# Autodesk Inventor assembly: main
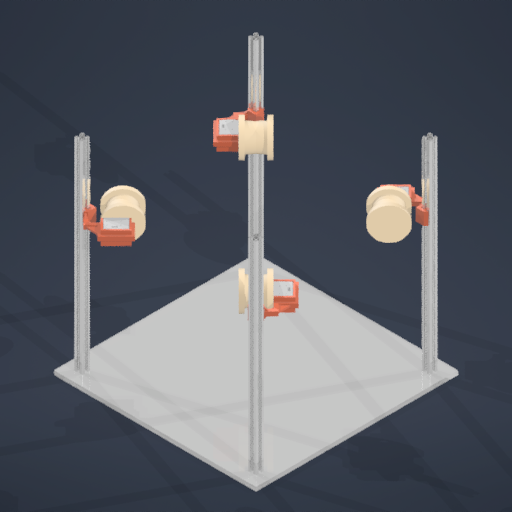
[picture p0: Inventor's stored thumbnail of the model, 512x512]
Saved by Autodesk Inventor 2026.2 (Build 302298010, 298A)
## iProperties
Created: 2026-02-11
Part Number: main
Document SubType Name: Assembly
Designer: Luke
Author: Luke
## Documents named in this file (3)
- C:\Users\Luke\OneDrive - Heriot-Watt University\Desktop\Robot Mech Sys\GroupProject\CAD\main.iam
- C:\Users\Luke\OneDrive - Heriot-Watt University\Desktop\Robot Mech Sys\GroupProject\CAD\parts\base.ipt
- C:\Users\Luke\OneDrive - Heriot-Watt University\Desktop\Robot Mech Sys\GroupProject\CAD\sub_assemblies\beam_sub_asssem.iam
## Components (5 placed, 2 different names)
1. base:1 — Mate:1, Mate:2, Mate:3, Flush:1, Flush:2
2. beam_sub_asssem:1 [sub-assembly] — Mate:1, Mate:2, Mate:3
3. beam_sub_asssem:2 [sub-assembly]
4. beam_sub_asssem:3 [sub-assembly]
5. beam_sub_asssem:4 [sub-assembly]
## Component patterns: (4 elements, first: beam_sub_asssem:1)
## Relationships (5: Mate 3, Flush 2)
- Mate:1: base:1 ↔ beam_sub_asssem:1
- Mate:2: base:1 ↔ beam_sub_asssem:1
- Mate:3: base:1 ↔ beam_sub_asssem:1
- Flush:1 (250 mm): base:1
- Flush:2 (250 mm): base:1
